# Autodesk Inventor assembly: _WandAssembly
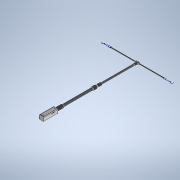
[picture p0: Inventor's stored thumbnail of the model, 180x180]
Saved by Autodesk Inventor 2022 (Build 260153000, 153)
## iProperties
Created: 2022-02-14
Part Number: _WandAssembly
Document SubType Name: Assembly
Designer: tecware
Author: tecware
## Documents named in this file (9)
- C:\Users\tecware\Documents\git\calibrationKit\calibrationKit_v1\T-wand\_WandAssembly.iam
- C:\Users\tecware\Documents\git\calibrationKit\calibrationKit_v1\T-wand\components_wand\T Clamp and Pipe Extension\Tclamp.ipt
- C:\Users\tecware\Documents\git\calibrationKit\calibrationKit_v1\T-wand\components_wand\verticalRodTop.ipt
- C:\Users\tecware\Documents\git\calibrationKit\calibrationKit_v1\T-wand\components_wand\horizontalRod.ipt
- C:\Users\tecware\Documents\git\calibrationKit\calibrationKit_v1\T-wand\components_wand\markerWithRodEnd.ipt
- C:\Users\tecware\Documents\git\calibrationKit\calibrationKit_v1\T-wand\Base Enclosure\_Enclosure Assembly.iam
- C:\Users\tecware\Documents\git\calibrationKit\calibrationKit_v1\T-wand\components_wand\T Clamp and Pipe Extension\pipeExtension.ipt
- C:\Users\tecware\Documents\git\calibrationKit\calibrationKit_v1\T-wand\components_wand\verticalRodBottom.ipt
- C:\Users\tecware\Documents\git\calibrationKit\calibrationKit_v1\LED Filament Assembly\LED Filament Assembly.iam
## Components (11 placed, 8 different names)
1. Tclamp:1 — Flush:1, Flush:2, Mate:5, Mate:6
2. verticalRodTop:1 — Flush:1, Mate:5, Mate:11, Mate:12
3. horizontalRod — Flush:2, Mate:6, Mate:7, Mate:8, Mate:9, Mate:10
4. markerWithRodEnd:1 — Mate:3, Mate:4, Flush:4, Mate:8, Mate:9
5. markerWithRodEnd:2 — Mate:3, Mate:4, Flush:4
6. markerWithRodEnd:3 — Mate:1, Flush:3, Mate:2, Mate:10
7. markerWithRodEnd:4 — Mate:1, Flush:3, Mate:2, Mate:7
8. _Enclosure Assembly:1 [sub-assembly] — Mate:15, Mate:16
9. pipeExtension:1 — Mate:11, Mate:12, Mate:13, Mate:14
10. verticalRodBottom:1 — Mate:13, Mate:14, Mate:15, Mate:16
11. LED Filament Assembly:1 [sub-assembly]
## Relationships (20: Mate 16, Flush 4)
- Flush:1: Tclamp:1 ↔ verticalRodTop:1
- Flush:2 (-15 mm): Tclamp:1 ↔ horizontalRod
- Mate:1: markerWithRodEnd:3 ↔ markerWithRodEnd:4
- Flush:3: markerWithRodEnd:3 ↔ markerWithRodEnd:4
- Mate:2: markerWithRodEnd:3 ↔ markerWithRodEnd:4
- Mate:3: markerWithRodEnd:1 ↔ markerWithRodEnd:2
- Mate:4: markerWithRodEnd:1 ↔ markerWithRodEnd:2
- Flush:4: markerWithRodEnd:1 ↔ markerWithRodEnd:2
- Mate:5: Tclamp:1 ↔ verticalRodTop:1
- Mate:6: Tclamp:1 ↔ horizontalRod
- Mate:7: horizontalRod ↔ markerWithRodEnd:4
- Mate:8: horizontalRod ↔ markerWithRodEnd:1
- Mate:9: horizontalRod ↔ markerWithRodEnd:1
- Mate:10: horizontalRod ↔ markerWithRodEnd:3
- Mate:11: verticalRodTop:1 ↔ pipeExtension:1
- Mate:12 (-20 mm): verticalRodTop:1 ↔ pipeExtension:1
- Mate:13: pipeExtension:1 ↔ verticalRodBottom:1
- Mate:14 (-20 mm): pipeExtension:1 ↔ verticalRodBottom:1
- Mate:15: _Enclosure Assembly:1 ↔ verticalRodBottom:1
- Mate:16 (-20 mm): _Enclosure Assembly:1 ↔ verticalRodBottom:1
